# Autodesk Inventor assembly: SHOULDER_v2
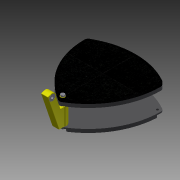
[picture p0: Inventor's stored thumbnail of the model, 180x180]
Saved by Autodesk Inventor 2014 (Build 180170000, 170)
## iProperties
Created: 2013-11-26
Part Number: SHOULDER_v2
Document SubType Name: Assembly
Designer: employee
Author: employee
## Documents named in this file (10)
- C:\Dev\Work\Drukarka\ConceptFORGE\GUS Simpson\INVENTOR FILES\SHOULDER_v2.iam
- C:\Dev\Work\Drukarka\ConceptFORGE\GUS Simpson\INVENTOR FILES\SHOULDER.ipt
- C:\Dev\Work\Drukarka\ConceptFORGE\GUS Simpson\INVENTOR FILES\_608.ipt
- C:\Dev\Work\Drukarka\ConceptFORGE\GUS Simpson\INVENTOR FILES\M8 WASHER.ipt
- C:\Dev\Work\Drukarka\ConceptFORGE\GUS Simpson\INVENTOR FILES\_BOTTOM PLATE.ipt
- C:\Dev\Work\Drukarka\ConceptFORGE\GUS Simpson\INVENTOR FILES\_TOP PLATE.ipt
- C:\Dev\Work\Drukarka\ConceptFORGE\GUS Simpson\INVENTOR FILES\M8 NUT.ipt
- C:\Dev\Work\Drukarka\ConceptFORGE\GUS Simpson\INVENTOR FILES\M8x100.ipt
- C:\Dev\Work\Drukarka\ConceptFORGE\GUS Simpson\INVENTOR FILES\PLASTIC WASHER.ipt
- C:\Dev\Work\Drukarka\ConceptFORGE\GUS Simpson\INVENTOR FILES\_BASALT BED.ipt
## Components (13 placed, 9 different names)
1. SHOULDER:1 — Insert:1, Insert:2, Insert:3, Insert:4
2. _608:1 — Insert:1
3. _608:2 — Insert:2
4. _608:3 — Insert:3, Insert:6
5. _608:4 — Insert:4, Insert:7
6. M8 WASHER:2 — Insert:6, Mate:2
7. M8 WASHER:3 — Insert:7, Mate:1
8. _BOTTOM PLATE:1 — Mate:1, Insert:9
9. _TOP PLATE:1 — Mate:2, Mate:5
10. M8 NUT:1 — Insert:9
11. M8x100:1 — Insert:8
12. PLASTIC WASHER:1 — Mate:6, Insert:8
13. _BASALT BED:1 — Mate:5, Mate:6
## Relationships (12: Insert 8, Mate 4)
- Insert:1: SHOULDER:1 ↔ _608:1
- Insert:2: SHOULDER:1 ↔ _608:2
- Insert:3: SHOULDER:1 ↔ _608:3
- Insert:4: SHOULDER:1 ↔ _608:4
- Insert:6: _608:3 ↔ M8 WASHER:2
- Insert:7: _608:4 ↔ M8 WASHER:3
- Mate:1: M8 WASHER:3 ↔ _BOTTOM PLATE:1
- Mate:2: M8 WASHER:2 ↔ _TOP PLATE:1
- Mate:5: _TOP PLATE:1 ↔ _BASALT BED:1
- Mate:6: PLASTIC WASHER:1 ↔ _BASALT BED:1
- Insert:8: M8x100:1 ↔ PLASTIC WASHER:1
- Insert:9: _BOTTOM PLATE:1 ↔ M8 NUT:1
